# Autodesk Inventor assembly: for_check
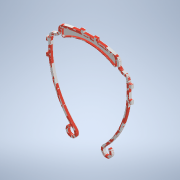
[picture p0: Inventor's stored thumbnail of the model, 180x180]
Saved by Autodesk Inventor 2020 (Build 240168000, 168)
## iProperties
Created: 2020-03-27
Part Number: for_check
Document SubType Name: Assembly
Designer: Clevo
Author: Clevo
## Documents named in this file (3)
- E:\Cornell_PPE_InjectionMolding\for_check.iam
- E:\Cornell_PPE_InjectionMolding\Visor_Frame_NORTH_AMERICA_V3.ipt
- E:\Cornell_PPE_InjectionMolding\headband.ipt
## Components (2 placed, 2 different names)
1. Visor_Frame_NORTH_AMERICA_V3:1 — Mate:1, Mate:2, Mate:3, Flush:1
2. headband:1 — Mate:1, Mate:2, Mate:3, Flush:1
## Relationships (4: Mate 3, Flush 1)
- Mate:1: Visor_Frame_NORTH_AMERICA_V3:1 ↔ headband:1
- Mate:2: Visor_Frame_NORTH_AMERICA_V3:1 ↔ headband:1
- Mate:3: Visor_Frame_NORTH_AMERICA_V3:1 ↔ headband:1
- Flush:1: Visor_Frame_NORTH_AMERICA_V3:1 ↔ headband:1
